# Autodesk Inventor assembly: vna_holder_v2
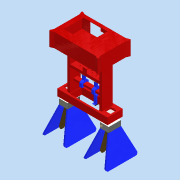
[picture p0: Inventor's stored thumbnail of the model, 180x180]
Saved by Autodesk Inventor 2022 (Build 260153000, 153)
## iProperties
Created: 2021-07-29
Part Number: vna_holder_v2
Document SubType Name: Assembly
Designer: nnico
Author: nnico
## Documents named in this file (16)
- C:\Users\nnico\Documents\Desminado Humanitario\Repositories\gpr20_vna_holder\assemblies\vna_holder.iam
- C:\Users\nnico\Documents\Desminado Humanitario\Repositories\gpr20_vna_holder\ipt\side_panel.ipt
- C:\Users\nnico\Documents\Desminado Humanitario\Repositories\gpr20_vna_holder\ipt\antennae_holder.ipt
- C:\Users\nnico\Documents\Desminado Humanitario\Repositories\gpr20_vna_holder\ipt\vna_mount.ipt
- C:\Users\nnico\Documents\Desminado Humanitario\Repositories\gpr20_vna_holder\ipt\vna_cover.ipt
- C:\Users\nnico\Documents\Desminado Humanitario\Repositories\gpr20_vna_holder\ipt\aux_strut.ipt
- C:\Users\nnico\Documents\Desminado Humanitario\Repositories\gpr20_vna_holder\ipt\aux_axis_support.ipt
- C:\Users\nnico\Documents\Desminado Humanitario\Repositories\gpr20_vna_holder\ipt\aux_axis_cap.ipt
- C:\Users\nnico\Documents\Desminado Humanitario\Repositories\gpr20_vna_holder\ipt\ir_sensor_support.ipt
- C:\Users\nnico\Documents\Desminado Humanitario\Repositories\gpr20_vna_holder\ipt\ir_sensor_cap.ipt
- C:\Users\nnico\Documents\Desminado Humanitario\Repositories\gpr20_vna_holder\assemblies\misc\IR Sharp sensor.iam
- C:\Users\nnico\Documents\Desminado Humanitario\Repositories\gpr20_vna_holder\assemblies\misc\NEMA17_MOTOR.ipt
- C:\Users\nnico\Documents\Desminado Humanitario\Repositories\gpr20_vna_holder\assemblies\misc\ANTENNA.ipt
- C:\Users\nnico\Documents\Desminado Humanitario\Repositories\gpr20_vna_holder\ipt\universal_mount.ipt
- C:\Users\nnico\Documents\Desminado Humanitario\Repositories\gpr20_vna_holder\assemblies\misc\SC12UU.ipt
- C:\Users\nnico\Documents\Desminado Humanitario\Repositories\gpr20_vna_holder\assemblies\misc\T8_NUT_HOUSING.ipt
## Components (21 placed, 15 different names)
1. side_panel:1 — Rigid:19
2. side_panel:2 — Rigid:3, Rigid:4, Rigid:10
3. antennae_holder:1 — Rigid:3, Mate:1, Mate:6, Mate:7, Flush:3, Rigid:15, Rigid:16
4. vna_mount:1 — Rigid:4, Rigid:9
5. vna_cover:1 — Rigid:9
6. aux_strut:1 — Rigid:10, Mate:2, Mate:3, Mate:4, Mate:5
7. aux_axis_support:1 — Rigid:11
8. aux_axis_support:2 — Rigid:12
9. aux_axis_cap:1 — Mate:2, Mate:3, Rigid:11
10. aux_axis_cap:2 — Mate:4, Mate:5, Rigid:12
11. ir_sensor_support:1 — Mate:6, Mate:7, Flush:3, Rigid:13, Rigid:14
12. ir_sensor_cap:1 — Rigid:13
13. IR Sharp sensor:1 [sub-assembly] — Rigid:14
14. NEMA17_MOTOR:1 — Rigid:15, Rigid:17
15. NEMA17_MOTOR:2 — Rigid:16, Rigid:18
16. ANTENNA:1 — Rigid:17
17. ANTENNA:2 — Rigid:18
18. universal_mount:1 — Rigid:19, Rigid:20, Rigid:21, Rigid:22
19. SC12UU:1 — Rigid:20
20. SC12UU:2 — Rigid:21
21. T8_NUT_HOUSING:1 — Rigid:22
## Relationships (24: WeldJoint 16, Mate 7, Flush 1)
- Rigid:3 [WeldJoint]: side_panel:2 ↔ antennae_holder:1
- Rigid:4 [WeldJoint]: side_panel:2 ↔ vna_mount:1
- Mate:1: antennae_holder:1
- Rigid:9 [WeldJoint]: vna_mount:1 ↔ vna_cover:1
- Rigid:10 [WeldJoint]: side_panel:2 ↔ aux_strut:1
- Mate:2: aux_strut:1 ↔ aux_axis_cap:1
- Mate:3: aux_strut:1 ↔ aux_axis_cap:1
- Rigid:11 [WeldJoint]: aux_axis_support:1 ↔ aux_axis_cap:1
- Mate:4: aux_strut:1 ↔ aux_axis_cap:2
- Mate:5: aux_strut:1 ↔ aux_axis_cap:2
- Rigid:12 [WeldJoint]: aux_axis_support:2 ↔ aux_axis_cap:2
- Mate:6: antennae_holder:1 ↔ ir_sensor_support:1
- Mate:7 (0.25 mm): antennae_holder:1 ↔ ir_sensor_support:1
- Flush:3 (-180 mm): antennae_holder:1 ↔ ir_sensor_support:1
- Rigid:13 [WeldJoint]: ir_sensor_support:1 ↔ ir_sensor_cap:1
- Rigid:14 [WeldJoint]: ir_sensor_support:1 ↔ IR Sharp sensor:1
- Rigid:15 [WeldJoint]: antennae_holder:1 ↔ NEMA17_MOTOR:1
- Rigid:16 [WeldJoint]: antennae_holder:1 ↔ NEMA17_MOTOR:2
- Rigid:17 [WeldJoint]: NEMA17_MOTOR:1 ↔ ANTENNA:1
- Rigid:18 [WeldJoint]: NEMA17_MOTOR:2 ↔ ANTENNA:2
- Rigid:19 [WeldJoint]: side_panel:1 ↔ universal_mount:1
- Rigid:20 [WeldJoint]: universal_mount:1 ↔ SC12UU:1
- Rigid:21 [WeldJoint]: universal_mount:1 ↔ SC12UU:2
- Rigid:22 [WeldJoint]: universal_mount:1 ↔ T8_NUT_HOUSING:1
